# Autodesk Inventor assembly: Ensamblaje2
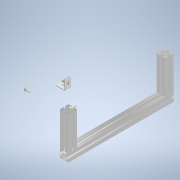
[picture p0: Inventor's stored thumbnail of the model, 180x180]
Saved by Autodesk Inventor 2021 (Build 250183000, 183)
## iProperties
Created: 2020-11-09
Part Number: Ensamblaje2
Document SubType Name: Assembly
Designer: juanm
Author: juanm
## Documents named in this file (5)
- C:\Users\juanm\OneDrive\Documentos\Inventor\NombreProyecto\Ensamblaje2.iam
- F:\CARRERA\INTERSEMESTRALES\RÓBOTICA\Rebot\Horizontal.ipt
- F:\CARRERA\INTERSEMESTRALES\RÓBOTICA\Rebot\Vertical.ipt
- F:\CARRERA\INTERSEMESTRALES\RÓBOTICA\Rebot\Tornillo.ipt
- F:\CARRERA\INTERSEMESTRALES\RÓBOTICA\Rebot\Sujetador2.ipt
## Components (6 placed, 4 different names)
1. Horizontal:1 — Nivelación:1, Nivelación:2, Coincidencia:1, Nivelación:3, Coincidencia:2, Nivelación:4
2. Vertical:1 — Nivelación:3, Coincidencia:2, Nivelación:4
3. Vertical:2 — Nivelación:1, Nivelación:2, Coincidencia:1, Nivelación:5, Coincidencia:3, Coincidencia:4
4. Tornillo:1
5. Tornillo:2 — Nivelación:5, Coincidencia:3, Coincidencia:4
6. Sujetador2:1
## Relationships (9: Flush 5, Mate 4)
- Nivelación:1 [Flush]: Horizontal:1 ↔ Vertical:2
- Nivelación:2 [Flush]: Horizontal:1 ↔ Vertical:2
- Coincidencia:1 [Mate]: Horizontal:1 ↔ Vertical:2
- Nivelación:3 [Flush]: Horizontal:1 ↔ Vertical:1
- Coincidencia:2 [Mate]: Horizontal:1 ↔ Vertical:1
- Nivelación:4 [Flush]: Horizontal:1 ↔ Vertical:1
- Nivelación:5 [Flush]: Vertical:2 ↔ Tornillo:2
- Coincidencia:3 [Mate]: Vertical:2 ↔ Tornillo:2
- Coincidencia:4 [Mate] (2.3 mm): Vertical:2 ↔ Tornillo:2
